# Autodesk Inventor assembly: Storage System Assembly
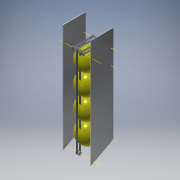
[picture p0: Inventor's stored thumbnail of the model, 180x180]
Saved by Autodesk Inventor 2019.4 (Build 234330000, 330)
## iProperties
Created: 2020-01-24
Part Number: Storage System Assembly
Document SubType Name: Assembly
Designer: admin
Author: admin
## Documents named in this file (9)
- C:\Users\admin\Desktop\FRC 2020 Engineering\GitHub\7738-2020\Robot V2\Storage System\Storage System Assembly.iam
- C:\Users\admin\Desktop\FRC 2020 Engineering\GitHub\7738-2020\Robot V2\Storage System\Storage Side Plate.ipt
- C:\Users\admin\Desktop\FRC 2020 Engineering\GitHub\7738-2020\Robot V2\Storage System\Storage System Assembly\Design Accelerator\Synchronous Belts Transmission1.iam
- C:\Users\admin\Desktop\FRC 2020 Engineering\GitHub\7738-2020\Robot V2\Storage System\Storage System Assembly\Design Accelerator\Synchronous Belts Transmission3.iam
- C:\Users\admin\Desktop\FRC 2020 Engineering\GitHub\7738-2020\Robot V2\Storage System\Storage System Assembly\Design Accelerator\Synchronous Belts Transmission4.iam
- C:\Users\admin\Desktop\FRC 2020 Engineering\GitHub\7738-2020\Robot V2\Storage System\Storage System Assembly\Design Accelerator\Synchronous Belts Transmission5.iam
- C:\Users\admin\Desktop\FRC 2020 Engineering\GitHub\7738-2020\Robot V2\Storage System\Storage System Assembly\Design Accelerator\Synchronous Belts Transmission6.iam
- C:\Users\admin\Desktop\FRC 2020 Engineering\GitHub\7738-2020\Power Cell.ipt
- C:\Users\admin\Desktop\FRC 2020 Engineering\GitHub\7738-2020\Robot V2\Turret\F6800.ipt
## Components (21 placed, 4 different names)
1. Storage Side Plate:1 — Mate:1, Mate:2, Mate:3, Flush:2, Mate:14, Mate:15, Mate:16, Mate:17, Mate:25, Mate:26, Mate:27, Mate:28, Mate:31, Mate:32
2. Storage Side Plate:2 — Mate:1, Mate:2, Flush:1, Mate:12, Mate:13, Mate:18, Mate:19, Mate:20, Mate:21, Mate:22, Mate:23, Mate:24, Mate:29, Mate:30
3. Synchronous Belts Transmission:1 [sub-assembly]
4. Synchronous Belts Transmission:2 [sub-assembly]
5. Synchronous Belts Transmission:3 [sub-assembly]
6. Synchronous Belts Transmission:4 [sub-assembly]
7. Synchronous Belts Transmission:5 [sub-assembly]
8. Power Cell:1 — Mate:4, Mate:8
9. Power Cell:2 — Mate:5, Mate:11
10. Power Cell:3 — Mate:6, Mate:9
11. Power Cell:4 — Mate:7, Mate:10
12. F6800:1 — Mate:13, Mate:24
13. F6800:2 — Mate:21, Mate:30
14. F6800:3 — Mate:19, Mate:22
15. F6800:4 — Mate:14, Mate:25
16. F6800:5 — Mate:15, Mate:26
17. F6800:7 — Mate:16, Mate:28
18. F6800:8 — Mate:17, Mate:27
19. F6800:9 — Mate:18, Mate:29
20. F6800:10 — Mate:20, Mate:23
21. F6800:11 — Mate:31, Mate:32
## Relationships (34: Mate 32, Flush 2)
- Mate:1: Storage Side Plate:1 ↔ Storage Side Plate:2
- Mate:2: Storage Side Plate:1 ↔ Storage Side Plate:2
- Mate:3 (114.3 mm): Storage Side Plate:1
- Flush:1 (114.3 mm): Storage Side Plate:2
- Mate:4: Power Cell:1
- Mate:5: Power Cell:2
- Mate:6: Power Cell:3
- Mate:7: Power Cell:4
- Mate:8: Power Cell:1
- Mate:9: Power Cell:3
- Mate:10: Power Cell:4
- Mate:11: Power Cell:2
- Mate:12: Storage Side Plate:2
- Flush:2: Storage Side Plate:1
- Mate:13: Storage Side Plate:2 ↔ F6800:1
- Mate:14: Storage Side Plate:1 ↔ F6800:4
- Mate:15: Storage Side Plate:1 ↔ F6800:5
- Mate:16: Storage Side Plate:1 ↔ F6800:7
- Mate:17: Storage Side Plate:1 ↔ F6800:8
- Mate:18: Storage Side Plate:2 ↔ F6800:9
- Mate:19: Storage Side Plate:2 ↔ F6800:3
- Mate:20: Storage Side Plate:2 ↔ F6800:10
- Mate:21: Storage Side Plate:2 ↔ F6800:2
- Mate:22 (0.2 mm): Storage Side Plate:2 ↔ F6800:3
- Mate:23 (0.2 mm): Storage Side Plate:2 ↔ F6800:10
- Mate:24 (0.2 mm): Storage Side Plate:2 ↔ F6800:1
- Mate:25 (0.2 mm): Storage Side Plate:1 ↔ F6800:4
- Mate:26 (0.2 mm): Storage Side Plate:1 ↔ F6800:5
- Mate:27 (0.2 mm): Storage Side Plate:1 ↔ F6800:8
- Mate:28 (0.2 mm): Storage Side Plate:1 ↔ F6800:7
- Mate:29 (0.2 mm): Storage Side Plate:2 ↔ F6800:9
- Mate:30 (0.2 mm): Storage Side Plate:2 ↔ F6800:2
- Mate:31: Storage Side Plate:1 ↔ F6800:11
- Mate:32 (0.2 mm): Storage Side Plate:1 ↔ F6800:11
